# Autodesk Inventor assembly: 3030_connector_assembled_MIR_MIR
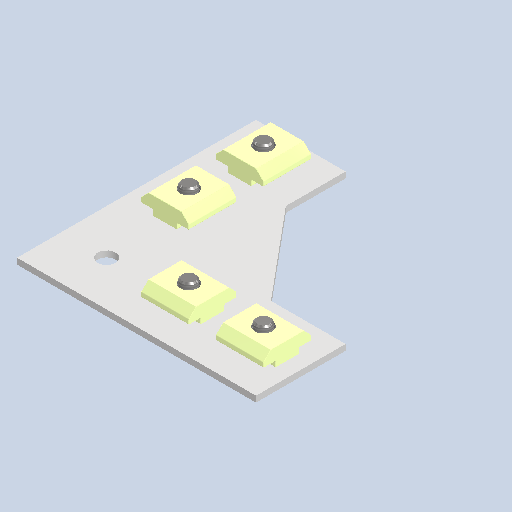
[picture p0: Inventor's stored thumbnail of the model, 512x512]
Saved by Autodesk Inventor 2024 (Build 280153000, 153)
## iProperties
Created: 2025-12-08
Part Number: 3030_connector_assembled_MIR_MIR
Document SubType Name: Assembly
Designer: schar
Author: schar
## Documents named in this file (4)
- C:\Users\schar\Desktop\projectBlueprint\AMSTS\hardware\3030_connector_assembled_MIR_MIR.iam
- C:\Users\schar\Desktop\projectBlueprint\AMSTS\hardware\Connect2x3030_m6_MIR_MIR.ipt
- C:\Users\schar\Desktop\projectBlueprint\AMSTS\hardware\3030_tnut_m6_MIR_MIR.ipt
- C:\Users\schar\Documents\Inventor\Content Center Files\R2024\en-US\AS 1420\AS 1420 - 1973 - M5 x 10.ipt
## Components (9 placed, 3 different names)
1. Connect2x3030_m6_MIR_MIR:1 — Insert:1, Insert:2, Insert:3, Insert:4, Rotational:4, Rotational:3, Rotational:1, Rotational:2
2. 3030_tnut_m6_MIR_MIR:1 — Rotational:4
3. 3030_tnut_m6_MIR_MIR:2 — Rotational:3
4. 3030_tnut_m6_MIR_MIR:3 — Rotational:1
5. 3030_tnut_m6_MIR_MIR:4 — Rotational:2
6. AS 1420 - Metric M5 x 10:1 — Insert:1
7. AS 1420 - Metric M5 x 10:2 — Insert:2
8. AS 1420 - Metric M5 x 10:3 — Insert:3
9. AS 1420 - Metric M5 x 10:4 — Insert:4
## Relationships (8: Insert 4, RevoluteJoint 4)
- Insert:1: Connect2x3030_m6_MIR_MIR:1 ↔ AS 1420 - Metric M5 x 10:1
- Insert:2: Connect2x3030_m6_MIR_MIR:1 ↔ AS 1420 - Metric M5 x 10:2
- Insert:3: Connect2x3030_m6_MIR_MIR:1 ↔ AS 1420 - Metric M5 x 10:3
- Insert:4: Connect2x3030_m6_MIR_MIR:1 ↔ AS 1420 - Metric M5 x 10:4
- Rotational:4 [RevoluteJoint] (-0.357 mm): Connect2x3030_m6_MIR_MIR:1 ↔ 3030_tnut_m6_MIR_MIR:1
- Rotational:3 [RevoluteJoint] (-0.357 mm): Connect2x3030_m6_MIR_MIR:1 ↔ 3030_tnut_m6_MIR_MIR:2
- Rotational:1 [RevoluteJoint] (-0.357 mm): Connect2x3030_m6_MIR_MIR:1 ↔ 3030_tnut_m6_MIR_MIR:3
- Rotational:2 [RevoluteJoint] (-0.357 mm): Connect2x3030_m6_MIR_MIR:1 ↔ 3030_tnut_m6_MIR_MIR:4
